# Autodesk Inventor assembly: frame
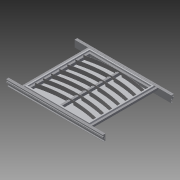
[picture p0: Inventor's stored thumbnail of the model, 180x180]
Saved by Autodesk Inventor 2013 (Build 170138000, 138)
## iProperties
Created: 2012-10-19
Part Number: frame
Document SubType Name: Assembly
Designer: Istvan
Mass: 30866 g
Surface Area: 132817 cm^2
Volume: 17609.3 cm^3
Density: 1.75282 g/cm^3
Author: Istvan
## Documents named in this file (4)
- C:\Users\istvan.burbank\Documents\GitHub\Crown-Fire\CAD\Frame\frame.iam
- C:\Users\istvan.burbank\Documents\GitHub\Crown-Fire\CAD\Frame\Table\table.iam
- C:\Users\istvan.burbank\Documents\GitHub\Crown-Fire\CAD\Frame\Supports\supports.iam
- C:\Users\istvan.burbank\Documents\GitHub\Crown-Fire\CAD\Frame\Table\rackRail.iam
## Components (4 placed, 3 different names)
1. supports:1 [sub-assembly] — Mate:30, Mate:33, Mate:34, Mate:35, Flush:18, Flush:19, Mate:36
2. table:1 [sub-assembly] — Mate:30, Mate:33, Mate:34, Mate:36
3. rackRail:1 [sub-assembly]
4. rackRail:2 [sub-assembly] — Mate:35, Flush:18, Flush:19
## Relationships (10: Mate 6, Flush 4)
- Mate:30: supports:1 ↔ table:1
- [Mate]: supports:1 ↔ rackRail:1
- [Flush]: supports:1 ↔ rackRail:1
- [Flush]: supports:1 ↔ rackRail:1
- Mate:33 (6.35 mm): supports:1 ↔ table:1
- Mate:34 (6.35 mm): supports:1 ↔ table:1
- Mate:35: supports:1 ↔ rackRail:2
- Flush:18: supports:1 ↔ rackRail:2
- Flush:19: supports:1 ↔ rackRail:2
- Mate:36: supports:1 ↔ table:1
